# Autodesk Inventor assembly: CameraEnclosure1
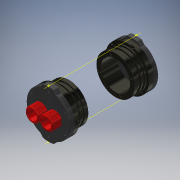
[picture p0: Inventor's stored thumbnail of the model, 180x180]
Saved by Autodesk Inventor 2018 (Build 220112000, 112)
## iProperties
Created: 2019-04-14
Part Number: CameraEnclosure1
Document SubType Name: Assembly
Designer: anirudh
Mass: 122.548 g
Surface Area: 729.678 cm^2
Volume: 122.548 cm^3
Density: 1 g/cm^3
Author: anirudh
## Documents named in this file (6)
- C:\Users\anirudh\Documents\MARS Fund\MATE Robotics\Silicon Sharks\2018-2019\CameraEnclosure\CameraEnclosure1.iam
- C:\Users\anirudh\Documents\MARS Fund\MATE Robotics\Silicon Sharks\2018-2019\CameraEnclosure\WTE2-M-END-CAP-2-HOLE-R1.ipt
- C:\Users\anirudh\Documents\MARS Fund\MATE Robotics\Silicon Sharks\2018-2019\CameraEnclosure\WTE2-M-END-CAP-R1.ipt
- C:\Users\anirudh\Documents\MARS Fund\MATE Robotics\Silicon Sharks\2018-2019\CameraEnclosure\WTE2-M-FLANGE-SEAL-R4.ipt
- C:\Users\anirudh\Documents\MARS Fund\MATE Robotics\Silicon Sharks\2018-2019\CameraEnclosure\WTE2-P-TUBE-12-R1.ipt
- C:\Users\anirudh\Documents\MARS Fund\MATE Robotics\Silicon Sharks\2018-2019\CameraEnclosure\6MMPenetrator.ipt
## Components (7 placed, 5 different names)
1. WTE2-M-END-CAP-2-HOLE-R1:1 — Mate:3, Mate:4, Mate:9, Mate:10, Mate:11, Mate:12, Mate:14, Mate:17, Mate:18, Mate:21
2. WTE2-M-END-CAP-R1:1 — Mate:7, Mate:8, Mate:15, Mate:16, Mate:19, Mate:20
3. WTE2-M-FLANGE-SEAL-R4:1 — Mate:5, Mate:6, Mate:7, Mate:8
4. WTE2-P-TUBE-12-R1:1 — Mate:1, Mate:2, Mate:5, Mate:6
5. WTE2-M-FLANGE-SEAL-R4:2 — Mate:1, Mate:2, Mate:3, Mate:4
6. 6MMPenetrator:1 — Mate:11, Mate:12
7. 6MMPenetrator:2 — Mate:9, Mate:10
## Relationships (20: Mate 20)
- Mate:1: WTE2-P-TUBE-12-R1:1 ↔ WTE2-M-FLANGE-SEAL-R4:2
- Mate:2: WTE2-P-TUBE-12-R1:1 ↔ WTE2-M-FLANGE-SEAL-R4:2
- Mate:3: WTE2-M-END-CAP-2-HOLE-R1:1 ↔ WTE2-M-FLANGE-SEAL-R4:2
- Mate:4: WTE2-M-END-CAP-2-HOLE-R1:1 ↔ WTE2-M-FLANGE-SEAL-R4:2
- Mate:5: WTE2-M-FLANGE-SEAL-R4:1 ↔ WTE2-P-TUBE-12-R1:1
- Mate:6: WTE2-M-FLANGE-SEAL-R4:1 ↔ WTE2-P-TUBE-12-R1:1
- Mate:7: WTE2-M-END-CAP-R1:1 ↔ WTE2-M-FLANGE-SEAL-R4:1
- Mate:8: WTE2-M-END-CAP-R1:1 ↔ WTE2-M-FLANGE-SEAL-R4:1
- Mate:9: WTE2-M-END-CAP-2-HOLE-R1:1 ↔ 6MMPenetrator:2
- Mate:10: WTE2-M-END-CAP-2-HOLE-R1:1 ↔ 6MMPenetrator:2
- Mate:11: WTE2-M-END-CAP-2-HOLE-R1:1 ↔ 6MMPenetrator:1
- Mate:12: WTE2-M-END-CAP-2-HOLE-R1:1 ↔ 6MMPenetrator:1
- Mate:14: WTE2-M-END-CAP-2-HOLE-R1:1
- Mate:15: WTE2-M-END-CAP-R1:1
- Mate:16: WTE2-M-END-CAP-R1:1
- Mate:17: WTE2-M-END-CAP-2-HOLE-R1:1
- Mate:18: WTE2-M-END-CAP-2-HOLE-R1:1
- Mate:19: WTE2-M-END-CAP-R1:1
- Mate:20: WTE2-M-END-CAP-R1:1
- Mate:21: WTE2-M-END-CAP-2-HOLE-R1:1
